# Autodesk Inventor assembly: przegub_3
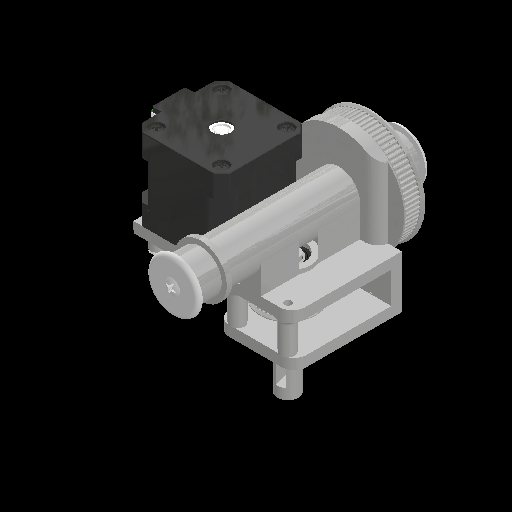
[picture p0: Inventor's stored thumbnail of the model, 512x512]
Saved by Autodesk Inventor 2024.4 (Build 284460000, 460)
## iProperties
Created: 2025-10-10
Part Number: przegub_3
Document SubType Name: Assembly
Designer: User
Mass: 157.32 g
Surface Area: 738.494 cm^2
Volume: 157.32 cm^3
Density: 1 g/cm^3
Author: User
## Documents named in this file (12)
- C:\Users\Duszy\Desktop\Projekty\Dummy\Dummy_v2\Model\Model\przegub_4\przegub_4.iam
- C:\Users\Duszy\Desktop\Projekty\Dummy\Dummy_v2\Model\Model\przegub_4\20_zb_wal.ipt
- C:\Users\Duszy\Desktop\Projekty\Dummy\Dummy_v2\Model\Model\przegub_4\5972K275_Ball Bearing.ipt
- C:\Users\Duszy\Desktop\Projekty\Dummy\Dummy_v2\Model\Model\przegub_4\Ankle_2.ipt
- C:\Users\Duszy\Desktop\Projekty\Dummy\Dummy_v2\Model\Model\przegub_4\m3-10mm_bc.ipt
- C:\Users\Duszy\Desktop\Projekty\Dummy\Dummy_v2\Model\Model\przegub_4\przeg-os-23.ipt
- C:\Users\Duszy\Desktop\Projekty\Dummy\Dummy_v2\Model\Model\przegub_4\przekladnia_40zb.ipt
- C:\Users\Duszy\Desktop\Projekty\Dummy\Dummy_v2\Model\Model\modele_gotowe\Modele_elementów\94459A769_Heat-Set Inserts for Plastic.ipt
- C:\Users\Duszy\Desktop\Projekty\Dummy\Dummy_v2\Model\Model\przegub_4\OBUD.ipt
- C:\Users\Duszy\Desktop\Projekty\Dummy\Dummy_v2\Model\Model\przegub_4\NEMA 17 Stepper Motor 39mm-NEMA 17 Stepper Motor 39mm.ipt
- C:\Users\Duszy\Desktop\Projekty\Dummy\Dummy_v2\Model\Model\przegub_4\m4-10mm.ipt
- C:\Users\Duszy\Desktop\Projekty\Dummy\Dummy_v2\Model\Model\przegub_4\94459A150_Heat-Set Inserts for Plastic.ipt
## Components (25 placed, 11 different names)
1. 20_zb_wal:1 — Obrotowe:6
2. 5972K275_Ball Bearing:1 — Obrotowe:2, Obrotowe:12
3. Ankle_2:1 — Obrotowe:1, Obrotowe:13
4. przeg-os-23:1 — Obrotowe:2, Sztywne:1, Obrotowe:4, Obrotowe:5, Obrotowe:7, Obrotowe:8, Obrotowe:11, Obrotowe:13
5. przekladnia_40zb:1 — Obrotowe:12
6. OBUD:1 — Obrotowe:11
7. 5972K275_Ball Bearing:2 — Obrotowe:1
8. NEMA 17 Stepper Motor 39mm-NEMA 17 Stepper Motor 39mm:1 — Sztywne:1, Obrotowe:3, Obrotowe:6
9. m4-10mm:1 — Obrotowe:10
10. 94459A150_Heat-Set Inserts for Plastic:2 — Obrotowe:4, Obrotowe:9, Sztywne:2
11. 94459A150_Heat-Set Inserts for Plastic:3 — Obrotowe:5, Obrotowe:10
12. m4-10mm:2 — Obrotowe:9
13. OBUD:2 — Sztywne:2
14. m3-10mm_bc:1 — Obrotowe:3
15. m3-10mm_bc:2
16. m3-10mm_bc:3
17. m3-10mm_bc:4
18. 94459A769_Heat-Set Inserts for Plastic:2 — Obrotowe:7, Obrotowe:15
19. 94459A769_Heat-Set Inserts for Plastic:3
20. 94459A769_Heat-Set Inserts for Plastic:1 — Obrotowe:8, Obrotowe:14
21. 94459A769_Heat-Set Inserts for Plastic:4
22. m3-10mm_bc:6 — Obrotowe:15
23. m3-10mm_bc:7
24. m3-10mm_bc:5 — Obrotowe:14
25. m3-10mm_bc:8
## Component patterns: (4 elements, first: m3-10mm_bc:1), (2 elements, first: 94459A769_Heat-Set Inserts for Plastic:2), (2 elements, first: 94459A769_Heat-Set Inserts for Plastic:1), (2 elements, first: m3-10mm_bc:6), (2 elements, first: m3-10mm_bc:5)
## Relationships (17: RevoluteJoint 15, WeldJoint 2)
- Obrotowe:1 [RevoluteJoint] (-5 mm): Ankle_2:1 ↔ 5972K275_Ball Bearing:2
- Obrotowe:2 [RevoluteJoint] (-5 mm): 5972K275_Ball Bearing:1 ↔ przeg-os-23:1
- Sztywne:1 [WeldJoint] (-5 mm): przeg-os-23:1 ↔ NEMA 17 Stepper Motor 39mm-NEMA 17 Stepper Motor 39mm:1
- Obrotowe:3 [RevoluteJoint] (2 mm): NEMA 17 Stepper Motor 39mm-NEMA 17 Stepper Motor 39mm:1 ↔ m3-10mm_bc:1
- Obrotowe:4 [RevoluteJoint]: przeg-os-23:1 ↔ 94459A150_Heat-Set Inserts for Plastic:2
- Obrotowe:5 [RevoluteJoint]: przeg-os-23:1 ↔ 94459A150_Heat-Set Inserts for Plastic:3
- Obrotowe:6 [RevoluteJoint]: 20_zb_wal:1 ↔ NEMA 17 Stepper Motor 39mm-NEMA 17 Stepper Motor 39mm:1
- Obrotowe:7 [RevoluteJoint]: przeg-os-23:1 ↔ 94459A769_Heat-Set Inserts for Plastic:2
- Obrotowe:8 [RevoluteJoint]: przeg-os-23:1 ↔ 94459A769_Heat-Set Inserts for Plastic:1
- Obrotowe:9 [RevoluteJoint] (-8 mm): 94459A150_Heat-Set Inserts for Plastic:2 ↔ m4-10mm:2
- Sztywne:2 [WeldJoint]: 94459A150_Heat-Set Inserts for Plastic:2 ↔ OBUD:2
- Obrotowe:10 [RevoluteJoint] (-8 mm): m4-10mm:1 ↔ 94459A150_Heat-Set Inserts for Plastic:3
- Obrotowe:11 [RevoluteJoint]: przeg-os-23:1 ↔ OBUD:1
- Obrotowe:12 [RevoluteJoint] (-0.8 mm): 5972K275_Ball Bearing:1 ↔ przekladnia_40zb:1
- Obrotowe:13 [RevoluteJoint]: Ankle_2:1 ↔ przeg-os-23:1
- Obrotowe:14 [RevoluteJoint] (-6 mm): 94459A769_Heat-Set Inserts for Plastic:1 ↔ m3-10mm_bc:5
- Obrotowe:15 [RevoluteJoint] (-6 mm): 94459A769_Heat-Set Inserts for Plastic:2 ↔ m3-10mm_bc:6
